# Autodesk Inventor assembly: SOIC-10 micro (RM-10)
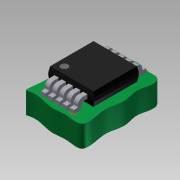
[picture p0: Inventor's stored thumbnail of the model, 180x180]
Saved by Autodesk Inventor 2011 (Build 150239000, 239)
## iProperties
Created: 2010-12-28
Part Number: SOIC-10 micro (RM-10)
Document SubType Name: Assembly
Designer: abbath
Mass: 0.0427566 g
Surface Area: 1.17417 cm^2
Volume: 0.0427566 cm^3
Density: 1 g/cm^3
Author: abbath
## Documents named in this file (3)
- D:\Abbath\Work\11.2\Сумматор light\КД\RSXX к сумматору\Установка элементов\SOIC-10 micro (RM-10) установка.iam
- D:\Abbath\Work\11.2\Сумматор light\КД\RSXX к сумматору\Установка элементов\SOIC-10 micro (RM-10).ipt
- D:\Abbath\Work\11.2\Сумматор light\КД\RSXX к сумматору\Установка элементов\SOIC-10 micro (RM-10) плата.ipt
## Components (2 placed, 2 different names)
1. SOIC-10 micro (RM-10):1 — Заподлицо:1, Заподлицо:2
2. SOIC-10 micro (RM-10) плата:1 — Заподлицо:1, Заподлицо:2
## Relationships (2: Flush 2)
- Заподлицо:1 [Flush]: SOIC-10 micro (RM-10):1 ↔ SOIC-10 micro (RM-10) плата:1
- Заподлицо:2 [Flush]: SOIC-10 micro (RM-10):1 ↔ SOIC-10 micro (RM-10) плата:1
